# Autodesk Inventor assembly: Assembly1
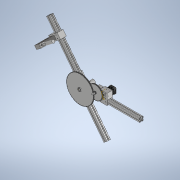
[picture p0: Inventor's stored thumbnail of the model, 180x180]
Saved by Autodesk Inventor 2022.3 (Build 263350000, 350)
## iProperties
Created: 2022-01-28
Part Number: Assembly1
Document SubType Name: Assembly
Designer: Martijn
Author: Martijn
## Documents named in this file (22)
- D:\phd\git\1dofsetup\Assembly1.iam
- D:\phd\git\1dofsetup\30x30x50.ipt
- D:\phd\git\1dofsetup\bearing_mount.ipt
- D:\phd\git\1dofsetup\NEMA 17.ipt
- D:\phd\git\1dofsetup\pololu-universal-aluminum-mounting-hub-for-5mm-shaft-m3-holes.ipt
- D:\phd\git\1dofsetup\space_plate.ipt
- D:\phd\git\1dofsetup\pololu-universal-aluminum-mounting-hub-for-8mm-shaft-m3-holes.ipt
- D:\phd\git\1dofsetup\SKF_608-2ZZ.ipt
- D:\phd\git\1dofsetup\load_cell.ipt
- D:\phd\git\1dofsetup\fixation_circle.ipt
- D:\phd\git\1dofsetup\fixation_plate2.ipt
- D:\phd\git\1dofsetup\8mm_to 6.35mm_kaplin.ipt
- D:\phd\git\1dofsetup\axis1.ipt
- D:\phd\git\1dofsetup\Lock Collar 8mm.ipt
- D:\phd\git\1dofsetup\bearing_mount3.ipt
- D:\phd\git\1dofsetup\axis2.ipt
- D:\phd\git\1dofsetup\loacell_mount1.ipt
- D:\phd\git\1dofsetup\big_gear.ipt
- D:\phd\git\1dofsetup\handle_vertical.ipt
- D:\phd\git\1dofsetup\double_gear.ipt
- D:\phd\git\1dofsetup\nema_mount.ipt
- D:\phd\git\1dofsetup\double_gear_mount.ipt
## Components (27 placed, 21 different names)
1. 30x30x50:1 — Mate:118, Flush:38, Mate:131, Flush:44, Mate:132, Mate:133, Mate:148, Flush:47, Mate:165, Flush:50
2. 30x30x50:2 — Mate:107, Mate:108, Flush:37, Flush:39, Mate:120, Flush:40, Mate:168, Mate:169, Mate:175, Mate:176
3. NEMA 17:1 — Mate:143, Mate:170, Mate:171, Mate:172, Mate:182
4. pololu-universal-aluminum-mounting-hub-for-5mm-shaft-m3-holes:1 — Mate:143, Mate:144, Mate:145, Mate:182, Mate:183
5. space_plate:1 — Flush:39, Mate:120, Flush:40, Mate:124, Flush:41, Flush:42
6. pololu-universal-aluminum-mounting-hub-for-8mm-shaft-m3-holes:1 — Flush:43, Mate:159, Mate:186, Mate:187
7. SKF_608-2ZZ:2 — Mate:136, Mate:179
8. SKF_608-2ZZ:4 — Mate:157, Mate:158
9. load_cell:1 — Mate:150, Mate:151, Mate:152, Mate:160, Mate:161, Flush:49
10. fixation_circle:1 — Mate:144, Mate:145, Mate:183
11. fixation_plate2:1 — Mate:118, Flush:38, Mate:122, Mate:125, Mate:126, Mate:133
12. 8mm_to 6.35mm_kaplin:1 — Mate:122, Mate:129
13. bearing_mount:1 — Mate:107, Mate:108, Flush:37, Mate:158
14. axis1:1 — Mate:77, Flush:30, Mate:136, Mate:174, Mate:184
15. Lock Collar 8mm:2 — Mate:77, Flush:30, Mate:178
16. bearing_mount3:1 — Mate:124, Flush:41, Flush:42, Mate:129, Mate:162, Mate:163
17. SKF_608-2ZZ:5 — Mate:125, Mate:126, Mate:162, Mate:163
18. axis2:1 — Flush:43, Mate:140, Mate:156, Mate:157, Mate:159
19. 30x30x50:3 — Mate:131, Flush:44, Mate:132, Mate:164
20. loacell_mount1:1 — Mate:148, Mate:150, Mate:151, Mate:152, Mate:165, Flush:50
21. big_gear:1 — Flush:47, Mate:156, Mate:164, Mate:173, Mate:186, Mate:187
22. handle_vertical:1 — Mate:160, Mate:161, Flush:49
23. double_gear:1 — Mate:173, Mate:174, Mate:177, Mate:185
24. nema_mount:1 — Mate:168, Mate:169, Mate:170, Mate:171, Mate:172
25. double_gear_mount:1 — Mate:175, Mate:176, Mate:177, Mate:178, Mate:179, Mate:180, Mate:181
26. SKF_608-2ZZ:6 — Mate:180, Mate:181
27. Lock Collar 8mm:3 — Mate:184, Mate:185
## Relationships (64: Mate 52, Flush 12)
- Mate:77: axis1:1 ↔ Lock Collar 8mm:2
- Flush:30 (0.5 mm): axis1:1 ↔ Lock Collar 8mm:2
- Mate:107: 30x30x50:2 ↔ bearing_mount:1
- Mate:108 (-30 mm): 30x30x50:2 ↔ bearing_mount:1
- Flush:37: 30x30x50:2 ↔ bearing_mount:1
- Mate:118: 30x30x50:1 ↔ fixation_plate2:1
- Flush:38: 30x30x50:1 ↔ fixation_plate2:1
- Flush:39: 30x30x50:2 ↔ space_plate:1
- Mate:120: 30x30x50:2 ↔ space_plate:1
- Flush:40: 30x30x50:2 ↔ space_plate:1
- Mate:122: fixation_plate2:1 ↔ 8mm_to 6.35mm_kaplin:1
- Mate:124: space_plate:1 ↔ bearing_mount3:1
- Flush:41: space_plate:1 ↔ bearing_mount3:1
- Flush:42: space_plate:1 ↔ bearing_mount3:1
- Mate:125: fixation_plate2:1 ↔ SKF_608-2ZZ:5
- Mate:126: fixation_plate2:1 ↔ SKF_608-2ZZ:5
- Flush:43: pololu-universal-aluminum-mounting-hub-for-8mm-shaft-m3-holes:1 ↔ axis2:1
- Mate:129 (5 mm): 8mm_to 6.35mm_kaplin:1 ↔ bearing_mount3:1
- Mate:131: 30x30x50:1 ↔ 30x30x50:3
- Flush:44: 30x30x50:1 ↔ 30x30x50:3
- Mate:132 (-60 mm): 30x30x50:1 ↔ 30x30x50:3
- Mate:133 (-60 mm): 30x30x50:1 ↔ fixation_plate2:1
- Mate:136: SKF_608-2ZZ:2 ↔ axis1:1
- Mate:140: axis2:1
- Mate:143: NEMA 17:1 ↔ pololu-universal-aluminum-mounting-hub-for-5mm-shaft-m3-holes:1
- Mate:144: pololu-universal-aluminum-mounting-hub-for-5mm-shaft-m3-holes:1 ↔ fixation_circle:1
- Mate:145: pololu-universal-aluminum-mounting-hub-for-5mm-shaft-m3-holes:1 ↔ fixation_circle:1
- Mate:148: 30x30x50:1 ↔ loacell_mount1:1
- Mate:150: load_cell:1 ↔ loacell_mount1:1
- Mate:151: load_cell:1 ↔ loacell_mount1:1
- Mate:152: load_cell:1 ↔ loacell_mount1:1
- Flush:47: 30x30x50:1 ↔ big_gear:1
- Mate:156: axis2:1 ↔ big_gear:1
- Mate:157: SKF_608-2ZZ:4 ↔ axis2:1
- Mate:158: SKF_608-2ZZ:4 ↔ bearing_mount:1
- Mate:159: pololu-universal-aluminum-mounting-hub-for-8mm-shaft-m3-holes:1 ↔ axis2:1
- Mate:160: load_cell:1 ↔ handle_vertical:1
- Mate:161: load_cell:1 ↔ handle_vertical:1
- Flush:49: load_cell:1 ↔ handle_vertical:1
- Mate:162: bearing_mount3:1 ↔ SKF_608-2ZZ:5
- Mate:163 (2 mm): bearing_mount3:1 ↔ SKF_608-2ZZ:5
- Mate:164: 30x30x50:3 ↔ big_gear:1
- Mate:165: 30x30x50:1 ↔ loacell_mount1:1
- Flush:50 (100 mm): 30x30x50:1 ↔ loacell_mount1:1
- Mate:168: 30x30x50:2 ↔ nema_mount:1
- Mate:169: 30x30x50:2 ↔ nema_mount:1
- Mate:170: NEMA 17:1 ↔ nema_mount:1
- Mate:171: NEMA 17:1 ↔ nema_mount:1
- Mate:172: NEMA 17:1 ↔ nema_mount:1
- Mate:173 (0.5 mm): big_gear:1 ↔ double_gear:1
- Mate:174: axis1:1 ↔ double_gear:1
- Mate:175: 30x30x50:2 ↔ double_gear_mount:1
- Mate:176: 30x30x50:2 ↔ double_gear_mount:1
- Mate:177: double_gear:1 ↔ double_gear_mount:1
- Mate:178: Lock Collar 8mm:2 ↔ double_gear_mount:1
- Mate:179: SKF_608-2ZZ:2 ↔ double_gear_mount:1
- Mate:180: double_gear_mount:1 ↔ SKF_608-2ZZ:6
- Mate:181: double_gear_mount:1 ↔ SKF_608-2ZZ:6
- Mate:182 (6.5 mm): NEMA 17:1 ↔ pololu-universal-aluminum-mounting-hub-for-5mm-shaft-m3-holes:1
- Mate:183: pololu-universal-aluminum-mounting-hub-for-5mm-shaft-m3-holes:1 ↔ fixation_circle:1
- Mate:184: axis1:1 ↔ Lock Collar 8mm:3
- Mate:185: double_gear:1 ↔ Lock Collar 8mm:3
- Mate:186: pololu-universal-aluminum-mounting-hub-for-8mm-shaft-m3-holes:1 ↔ big_gear:1
- Mate:187: pololu-universal-aluminum-mounting-hub-for-8mm-shaft-m3-holes:1 ↔ big_gear:1
